# Autodesk Inventor assembly: Fr.wing_assy
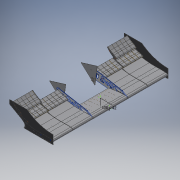
[picture p0: Inventor's stored thumbnail of the model, 180x180]
Saved by Autodesk Inventor 2018.2 (Build 222227000, 227)
## iProperties
Created: 2018-03-05
Part Number: Fr.wing_assy
Material: 一般
Document SubType Name: Assembly
Designer: ku_sk
Mass: 11232.8 g
Surface Area: 27769.7 cm^2
Volume: 11454.5 cm^3
Density: 0.980642 g/cm^3
Author: ku_sk
## Documents named in this file (13)
- C:\Users\ku_sk\Documents\Inventor\Aero\KS-15\Fr.wing\Fr.wing_assy.iam
- C:\Users\ku_sk\Documents\Inventor\Aero\KS-15\Fr.wing\parts\mainflap_side\mainflap_side.iam
- C:\Users\ku_sk\Documents\Inventor\Aero\KS-15\Fr.wing\parts\mainflap_center\mainflap_center.iam
- C:\Users\ku_sk\Documents\Inventor\Aero\KS-15\Fr.wing\parts\subflap\subflap.iam
- C:\Users\ku_sk\Documents\Inventor\Aero\KS-15\Fr.wing\parts\bracket1\bracket1.ipt
- C:\Users\ku_sk\Documents\Inventor\Aero\KS-15\Fr.wing\parts\bracket2.ipt
- C:\Users\ku_sk\Documents\Inventor\Aero\KS-15\Fr.wing\parts\endplate.ipt
- C:\Users\ku_sk\Documents\Inventor\Aero\KS-15\Fr.wing\parts\endplate1.ipt
- C:\Users\ku_sk\Documents\Inventor\Aero\KS-15\Fr.wing\bracket1(body).ipt
- C:\Users\ku_sk\Documents\Inventor\Aero\KS-15\Fr.wing\parts\axis_f3.ipt
- C:\Users\ku_sk\Documents\Inventor\Aero\KS-15\Fr.wing\parts\axis_f2.ipt
- C:\Users\ku_sk\Documents\Inventor\Aero\KS-15\Fr.wing\parts\axis_f1.ipt
- C:\Users\ku_sk\Documents\Inventor\Aero\KS-15\Fr.wing\mount2.ipt
## Components (31 placed, 12 different names)
1. mainflap_center:1 [sub-assembly] — フラッシュ:1, メイト:1, メイト:4, メイト:5, メイト:6, メイト:7, 角度:1, メイト:50, メイト:51, メイト:52, メイト:53, メイト:54, メイト:55
2. mainflap_side:1 [sub-assembly] — メイト:4, メイト:7, メイト:8, メイト:9, メイト:10, フラッシュ:2, メイト:46, メイト:56, メイト:57, メイト:64
3. mainflap_side:2 [sub-assembly] — メイト:5, メイト:6, メイト:11, メイト:12, メイト:13, フラッシュ:4, メイト:49, メイト:65
4. mainflap_side:3 [sub-assembly] — メイト:8, メイト:9, メイト:10, フラッシュ:3, メイト:45, メイト:78, メイト:79, フラッシュ:20
5. mainflap_side:4 [sub-assembly] — メイト:11, メイト:12, メイト:13, フラッシュ:5, メイト:44
6. subflap:1 [sub-assembly] — メイト:14, メイト:15, メイト:19, フラッシュ:2, メイト:20, メイト:21, メイト:58, メイト:59
7. subflap:2 [sub-assembly] — メイト:14, メイト:15, メイト:19, フラッシュ:3, フラッシュ:7
8. subflap:3 [sub-assembly] — メイト:22, メイト:23, フラッシュ:7, メイト:60, メイト:61
9. subflap:4 [sub-assembly] — メイト:16, メイト:17, メイト:18, フラッシュ:4, メイト:20, メイト:21, メイト:63
10. subflap:5 [sub-assembly] — メイト:16, メイト:17, メイト:18, フラッシュ:5, フラッシュ:6, メイト:76, フラッシュ:18, メイト:77
11. subflap:6 [sub-assembly] — メイト:22, メイト:23, フラッシュ:6, メイト:62
12. endplate:1 — メイト:44, フラッシュ:8, フラッシュ:9
13. endplate1:1 — メイト:45, フラッシュ:8, フラッシュ:9
14. bracket2:1 — メイト:46, メイト:56, メイト:57, メイト:58, メイト:59, メイト:60, メイト:61, メイト:72, メイト:73, フラッシュ:14
15. bracket2:2 — メイト:49, メイト:62, メイト:63, メイト:70, メイト:71, フラッシュ:12
16. bracket1:1 — メイト:52, メイト:53, メイト:54, メイト:65, メイト:66, メイト:69, メイト:80, メイト:81
17. bracket1:2 — メイト:50, メイト:51, メイト:55, メイト:64, メイト:67, メイト:68, メイト:74, メイト:75, フラッシュ:16, メイト:82, メイト:83
18. bracket1(body):1 — メイト:66, メイト:69, フラッシュ:10, 角度:2
19. bracket1(body):2 — メイト:67, メイト:68, フラッシュ:10
20. axis_f3:1 — フラッシュ:11, メイト:71
21. axis_f3:2 — フラッシュ:11, メイト:70, フラッシュ:12
22. axis_f3:3 — フラッシュ:13, メイト:73
23. axis_f3:4 — フラッシュ:13, メイト:72, フラッシュ:14
24. axis_f2:1 — フラッシュ:17, メイト:77
25. axis_f2:2 — フラッシュ:17, メイト:76, フラッシュ:18
26. axis_f2:3 — フラッシュ:15, メイト:75, フラッシュ:16
27. axis_f2:4 — フラッシュ:15, メイト:74
28. axis_f1:1 — フラッシュ:19, メイト:79
29. axis_f1:2 — フラッシュ:19, メイト:78, フラッシュ:20
30. mount2:1 — メイト:80, メイト:81, フラッシュ:21
31. mount2:2 — メイト:82, メイト:83, フラッシュ:21
## Relationships (82: Mate 59, Flush 21, Angle 2)
- フラッシュ:1 [Flush]: mainflap_center:1
- メイト:1 [Mate]: mainflap_center:1
- メイト:4 [Mate]: mainflap_center:1 ↔ mainflap_side:1
- メイト:5 [Mate]: mainflap_center:1 ↔ mainflap_side:2
- メイト:6 [Mate]: mainflap_center:1 ↔ mainflap_side:2
- メイト:7 [Mate]: mainflap_center:1 ↔ mainflap_side:1
- メイト:8 [Mate] (4 mm): mainflap_side:1 ↔ mainflap_side:3
- メイト:9 [Mate]: mainflap_side:1 ↔ mainflap_side:3
- メイト:10 [Mate]: mainflap_side:1 ↔ mainflap_side:3
- メイト:11 [Mate] (4 mm): mainflap_side:2 ↔ mainflap_side:4
- メイト:12 [Mate]: mainflap_side:2 ↔ mainflap_side:4
- メイト:13 [Mate]: mainflap_side:2 ↔ mainflap_side:4
- メイト:14 [Mate]: subflap:1 ↔ subflap:2
- メイト:15 [Mate]: subflap:1 ↔ subflap:2
- メイト:16 [Mate] (4 mm): subflap:4 ↔ subflap:5
- メイト:17 [Mate]: subflap:4 ↔ subflap:5
- メイト:18 [Mate]: subflap:4 ↔ subflap:5
- メイト:19 [Mate] (4 mm): subflap:1 ↔ subflap:2
- フラッシュ:2 [Flush]: mainflap_side:1 ↔ subflap:1
- フラッシュ:3 [Flush]: mainflap_side:3 ↔ subflap:2
- フラッシュ:4 [Flush]: mainflap_side:2 ↔ subflap:4
- フラッシュ:5 [Flush]: mainflap_side:4 ↔ subflap:5
- メイト:20 [Mate]: subflap:1 ↔ subflap:4
- メイト:21 [Mate]: subflap:1 ↔ subflap:4
- メイト:22 [Mate]: subflap:3 ↔ subflap:6
- メイト:23 [Mate]: subflap:3 ↔ subflap:6
- フラッシュ:6 [Flush]: subflap:5 ↔ subflap:6
- フラッシュ:7 [Flush]: subflap:2 ↔ subflap:3
- メイト:44 [Mate]: mainflap_side:4 ↔ endplate:1
- メイト:45 [Mate]: mainflap_side:3 ↔ endplate1:1
- フラッシュ:8 [Flush]: endplate:1 ↔ endplate1:1
- フラッシュ:9 [Flush]: endplate:1 ↔ endplate1:1
- 角度:1 [Angle] (4 deg): mainflap_center:1
- メイト:46 [Mate]: mainflap_side:1 ↔ bracket2:1
- メイト:49 [Mate]: mainflap_side:2 ↔ bracket2:2
- メイト:50 [Mate]: mainflap_center:1 ↔ bracket1:2
- メイト:51 [Mate]: mainflap_center:1 ↔ bracket1:2
- メイト:52 [Mate]: mainflap_center:1 ↔ bracket1:1
- メイト:53 [Mate]: mainflap_center:1 ↔ bracket1:1
- メイト:54 [Mate]: mainflap_center:1 ↔ bracket1:1
- メイト:55 [Mate]: mainflap_center:1 ↔ bracket1:2
- メイト:56 [Mate]: mainflap_side:1 ↔ bracket2:1
- メイト:57 [Mate]: mainflap_side:1 ↔ bracket2:1
- メイト:58 [Mate]: subflap:1 ↔ bracket2:1
- メイト:59 [Mate]: subflap:1 ↔ bracket2:1
- メイト:60 [Mate]: subflap:3 ↔ bracket2:1
- メイト:61 [Mate]: subflap:3 ↔ bracket2:1
- メイト:62 [Mate]: subflap:6 ↔ bracket2:2
- メイト:63 [Mate]: subflap:4 ↔ bracket2:2
- メイト:64 [Mate]: mainflap_side:1 ↔ bracket1:2
- メイト:65 [Mate]: mainflap_side:2 ↔ bracket1:1
- メイト:66 [Mate]: bracket1:1 ↔ bracket1(body):1
- メイト:67 [Mate]: bracket1:2 ↔ bracket1(body):2
- メイト:68 [Mate] (5 mm): bracket1:2 ↔ bracket1(body):2
- メイト:69 [Mate] (5 mm): bracket1:1 ↔ bracket1(body):1
- フラッシュ:10 [Flush]: bracket1(body):1 ↔ bracket1(body):2
- 角度:2 [Angle] (0 deg): bracket1(body):1
- フラッシュ:11 [Flush]: axis_f3:1 ↔ axis_f3:2
- メイト:70 [Mate]: bracket2:2 ↔ axis_f3:2
- メイト:71 [Mate]: bracket2:2 ↔ axis_f3:1
- フラッシュ:12 [Flush]: bracket2:2 ↔ axis_f3:2
- フラッシュ:13 [Flush]: axis_f3:3 ↔ axis_f3:4
- メイト:72 [Mate]: bracket2:1 ↔ axis_f3:4
- メイト:73 [Mate]: bracket2:1 ↔ axis_f3:3
- フラッシュ:14 [Flush]: bracket2:1 ↔ axis_f3:4
- フラッシュ:15 [Flush]: axis_f2:3 ↔ axis_f2:4
- メイト:74 [Mate]: bracket1:2 ↔ axis_f2:4
- メイト:75 [Mate]: bracket1:2 ↔ axis_f2:3
- フラッシュ:16 [Flush]: bracket1:2 ↔ axis_f2:3
- フラッシュ:17 [Flush]: axis_f2:1 ↔ axis_f2:2
- メイト:76 [Mate]: subflap:5 ↔ axis_f2:2
- フラッシュ:18 [Flush]: subflap:5 ↔ axis_f2:2
- メイト:77 [Mate]: subflap:5 ↔ axis_f2:1
- フラッシュ:19 [Flush]: axis_f1:1 ↔ axis_f1:2
- メイト:78 [Mate]: mainflap_side:3 ↔ axis_f1:2
- メイト:79 [Mate]: mainflap_side:3 ↔ axis_f1:1
- フラッシュ:20 [Flush]: mainflap_side:3 ↔ axis_f1:2
- メイト:80 [Mate]: bracket1:1 ↔ mount2:1
- メイト:81 [Mate] (10 mm): bracket1:1 ↔ mount2:1
- メイト:82 [Mate]: bracket1:2 ↔ mount2:2
- メイト:83 [Mate] (10 mm): bracket1:2 ↔ mount2:2
- フラッシュ:21 [Flush]: mount2:1 ↔ mount2:2
